# Autodesk Inventor assembly: j1 assmble
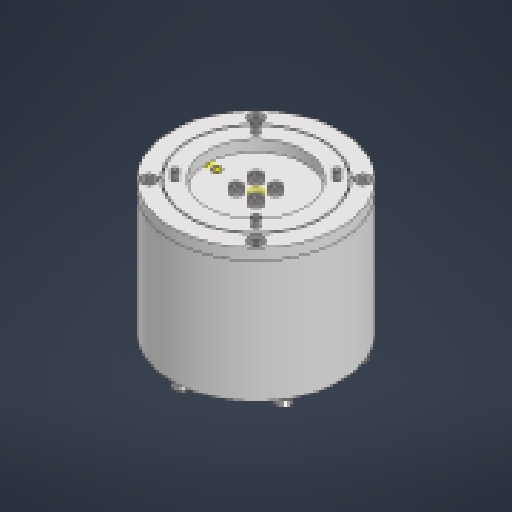
[picture p0: Inventor's stored thumbnail of the model, 512x512]
Saved by Autodesk Inventor 2026.2 (Build 302298000, 298)
## iProperties
Created: 2025-07-11
Part Number: j1 assmble
Document SubType Name: Assembly
Designer: gavin
Author: gavin
## Documents named in this file (15)
- D:\Github\6-DOF-Robot-Arm\3D-model\robot armT 2(CAD file)\j1 assmble.iam
- D:\Github\6-DOF-Robot-Arm\3D-model\robot armT 2(CAD file)\arm bearing.ipt
- D:\Github\6-DOF-Robot-Arm\3D-model\robot armT 2(CAD file)\nema23_57HS56.ipt
- D:\Github\6-DOF-Robot-Arm\3D-model\robot armT 2(CAD file)\xl28 driven.ipt
- D:\Github\6-DOF-Robot-Arm\3D-model\robot armT 2(CAD file)\j1 moving plate.ipt
- D:\Github\6-DOF-Robot-Arm\3D-model\robot armT 2(CAD file)\j1 57 mount.ipt
- D:\Github\6-DOF-Robot-Arm\3D-model\robot armT 2(CAD file)\optic endstop module.ipt
- D:\Github\6-DOF-Robot-Arm\3D-model\robot armT 2(CAD file)\DIN 7991 - M5x12.ipt
- D:\Github\6-DOF-Robot-Arm\3D-model\robot armT 2(CAD file)\CNS 4557 - M5 x 0.8 x 10.ipt
- D:\Github\6-DOF-Robot-Arm\3D-model\robot armT 2(CAD file)\DIN 7991 - M5x20.ipt
- D:\Github\6-DOF-Robot-Arm\3D-model\robot armT 2(CAD file)\j1 endstop block v2.ipt
- D:\Github\6-DOF-Robot-Arm\3D-model\robot armT 2(CAD file)\BS 4168 - M5 x 16(7).ipt
- D:\Github\6-DOF-Robot-Arm\3D-model\robot armT 2(CAD file)\M5 heat set inserts.ipt
- D:\Github\6-DOF-Robot-Arm\3D-model\robot armT 2(CAD file)\AS 1427 - M3 x 6(5) II.ipt
- D:\Github\6-DOF-Robot-Arm\3D-model\robot armT 2(CAD file)\CNS 4558 - M3 x 0.5 x 10.ipt
## Components (42 placed, 14 different names)
1. arm bearing:1
2. nema23_57HS56:1
3. xl28 driven:1
4. j1 moving plate:1 — 齊平:4, 剛性:13
5. j1 57 mount:1 — 剛性:1, 剛性:2, 剛性:3, 剛性:4, 剛性:5, 剛性:6, 剛性:7, 剛性:8, 剛性:9, 剛性:10, 旋轉:13, 旋轉:14, 旋轉:15, 旋轉:16
6. optic endstop module:1 — 剛性:11, 剛性:12
7. DIN 7991 - M5x12:1
8. DIN 7991 - M5x12:2
9. DIN 7991 - M5x12:3
10. DIN 7991 - M5x12:4
11. DIN 7991 - M5x12:5
12. DIN 7991 - M5x12:6
13. DIN 7991 - M5x12:7
14. DIN 7991 - M5x12:8
15. DIN 7991 - M5x12:9
16. DIN 7991 - M5x12:10
17. CNS 4557 - M5 x 0.8 x 10:1
18. CNS 4557 - M5 x 0.8 x 10:2
19. CNS 4557 - M5 x 0.8 x 10:3
20. CNS 4557 - M5 x 0.8 x 10:4
21. DIN 7991 - M5x20:1
22. DIN 7991 - M5x20:2
23. DIN 7991 - M5x20:3
24. DIN 7991 - M5x20:4
25. j1 endstop block v2:1 — 齊平:4
26. BS 4168 - M5 x 16(7):1 — 旋轉:13
27. BS 4168 - M5 x 16(7):2 — 旋轉:15
28. BS 4168 - M5 x 16(7):3 — 旋轉:14
29. BS 4168 - M5 x 16(7):4 — 旋轉:16
30. M5 heat set inserts:1 — 剛性:7
31. M5 heat set inserts:2 — 剛性:10
32. M5 heat set inserts:3 — 剛性:8
33. M5 heat set inserts:4 — 剛性:4
34. M5 heat set inserts:5 — 剛性:9
35. M5 heat set inserts:6 — 剛性:6
36. M5 heat set inserts:7 — 剛性:1
37. M5 heat set inserts:8 — 剛性:5
38. M5 heat set inserts:9 — 剛性:3
39. M5 heat set inserts:10 — 剛性:2
40. AS 1427 - M3 x 6(5) II:1 — 剛性:11
41. AS 1427 - M3 x 6(5) II:2 — 剛性:12
42. CNS 4558 - M3 x 0.5 x 10:1 — 剛性:13
## Relationships (47: RevoluteJoint 16, Mate 14, WeldJoint 13, Flush 4)
- [Mate]: arm bearing:1 ↔ j1 moving plate:1
- [Mate]: arm bearing:1 ↔ j1 moving plate:1
- [Mate]: arm bearing:1 ↔ j1 moving plate:1
- [Mate]: xl28 driven:1 ↔ j1 moving plate:1
- [Mate]: xl28 driven:1 ↔ j1 moving plate:1
- [Mate]: xl28 driven:1 ↔ j1 moving plate:1
- [Mate]: nema23_57HS56:1 ↔ xl28 driven:1
- [Mate]: nema23_57HS56:1 ↔ xl28 driven:1
- [Flush]: nema23_57HS56:1 ↔ j1 57 mount:1
- [Flush]: nema23_57HS56:1 ↔ j1 57 mount:1
- [Flush]: nema23_57HS56:1 ↔ j1 57 mount:1
- [Mate]: nema23_57HS56:1 ↔ j1 57 mount:1
- [Mate]: arm bearing:1 ↔ j1 57 mount:1
- [Mate]: arm bearing:1 ↔ j1 57 mount:1
- [Mate]: j1 57 mount:1 ↔ optic endstop module:1
- [Mate]: j1 57 mount:1 ↔ optic endstop module:1
- [Mate]: j1 57 mount:1 ↔ optic endstop module:1
- [RevoluteJoint]: arm bearing:1 ↔ DIN 7991 - M5x12:1
- [RevoluteJoint]: arm bearing:1 ↔ DIN 7991 - M5x12:6
- [RevoluteJoint]: arm bearing:1 ↔ DIN 7991 - M5x12:5
- [RevoluteJoint]: arm bearing:1 ↔ DIN 7991 - M5x12:2
- [RevoluteJoint]: j1 moving plate:1 ↔ CNS 4557 - M5 x 0.8 x 10:1
- [RevoluteJoint]: j1 moving plate:1 ↔ CNS 4557 - M5 x 0.8 x 10:2
- [RevoluteJoint]: j1 moving plate:1 ↔ CNS 4557 - M5 x 0.8 x 10:3
- [RevoluteJoint]: j1 moving plate:1 ↔ CNS 4557 - M5 x 0.8 x 10:4
- [RevoluteJoint]: j1 moving plate:1 ↔ DIN 7991 - M5x20:1
- [RevoluteJoint]: j1 moving plate:1 ↔ DIN 7991 - M5x20:2
- [RevoluteJoint]: j1 moving plate:1 ↔ DIN 7991 - M5x20:3
- [RevoluteJoint]: j1 moving plate:1 ↔ DIN 7991 - M5x20:4
- 齊平:4 [Flush]: j1 moving plate:1 ↔ j1 endstop block v2:1
- 剛性:1 [WeldJoint]: j1 57 mount:1 ↔ M5 heat set inserts:7
- 剛性:2 [WeldJoint]: j1 57 mount:1 ↔ M5 heat set inserts:10
- 剛性:3 [WeldJoint]: j1 57 mount:1 ↔ M5 heat set inserts:9
- 剛性:4 [WeldJoint]: j1 57 mount:1 ↔ M5 heat set inserts:4
- 剛性:5 [WeldJoint]: j1 57 mount:1 ↔ M5 heat set inserts:8
- 剛性:6 [WeldJoint]: j1 57 mount:1 ↔ M5 heat set inserts:6
- 剛性:7 [WeldJoint]: j1 57 mount:1 ↔ M5 heat set inserts:1
- 剛性:8 [WeldJoint]: j1 57 mount:1 ↔ M5 heat set inserts:3
- 剛性:9 [WeldJoint]: j1 57 mount:1 ↔ M5 heat set inserts:5
- 剛性:10 [WeldJoint]: j1 57 mount:1 ↔ M5 heat set inserts:2
- 剛性:11 [WeldJoint]: optic endstop module:1 ↔ AS 1427 - M3 x 6(5) II:1
- 剛性:12 [WeldJoint]: optic endstop module:1 ↔ AS 1427 - M3 x 6(5) II:2
- 剛性:13 [WeldJoint]: j1 moving plate:1 ↔ CNS 4558 - M3 x 0.5 x 10:1
- 旋轉:13 [RevoluteJoint]: j1 57 mount:1 ↔ BS 4168 - M5 x 16(7):1
- 旋轉:14 [RevoluteJoint]: j1 57 mount:1 ↔ BS 4168 - M5 x 16(7):3
- 旋轉:15 [RevoluteJoint]: j1 57 mount:1 ↔ BS 4168 - M5 x 16(7):2
- 旋轉:16 [RevoluteJoint]: j1 57 mount:1 ↔ BS 4168 - M5 x 16(7):4
## Named parameters: d34_d40 = 0 mm, d35_d41 = 0 mm
